# Autodesk Inventor assembly: nc_nhk20
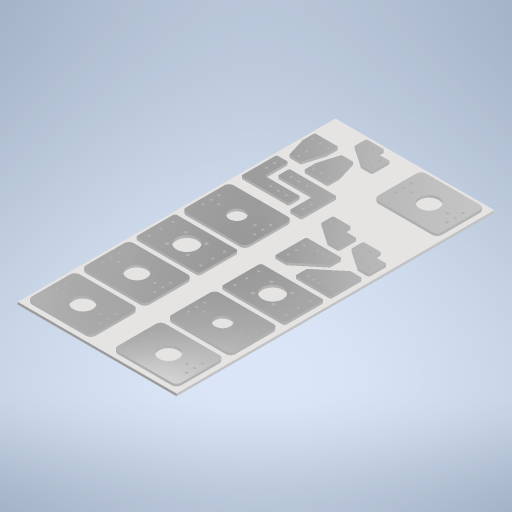
[picture p0: Inventor's stored thumbnail of the model, 512x512]
Saved by Autodesk Inventor 2023 (Build 270158000, 158)
## iProperties
Created: 2022-04-28
Part Number: nc_nhk20
Document SubType Name: Assembly
Designer: yuta
Author: yuta
## Documents named in this file (9)
- C:\Users\yuta\Documents\NHK\nc_nhk20.iam
- C:\Users\yuta\Documents\NHK\NC.port.ipt
- C:\Users\yuta\Documents\NHK\射出_エンコーダー固定.ipt
- C:\Users\yuta\Documents\NHK\射出_エンコーダー固定2.ipt
- C:\Users\yuta\Documents\NHK\射出_モーター固定1.ipt
- C:\Users\yuta\Documents\NHK\射出_固定3.ipt
- C:\Users\yuta\Documents\NHK\射出_固定6.ipt
- C:\Users\yuta\Documents\NHK\射出_固定5.ipt
- C:\Users\yuta\Documents\NHK\射出_固定4.ipt
## Components (18 placed, 8 different names)
1. NC.port:1 — メイト:1, フラッシュ:1, フラッシュ:2, メイト:2, フラッシュ:3, フラッシュ:4, メイト:3, フラッシュ:5, メイト:5, フラッシュ:6, メイト:7, フラッシュ:7, メイト:9, フラッシュ:8, メイト:11, フラッシュ:9, メイト:13, フラッシュ:10, メイト:15, メイト:20, フラッシュ:12, メイト:23, フラッシュ:14, メイト:26, フラッシュ:15, フラッシュ:16, メイト:27, フラッシュ:17, メイト:29, メイト:32, フラッシュ:18, フラッシュ:19
2. 射出_エンコーダー固定:1 — メイト:1, フラッシュ:1, フラッシュ:2, メイト:4
3. 射出_エンコーダー固定:2 — メイト:2, フラッシュ:3, フラッシュ:4, メイト:6
4. 射出_エンコーダー固定:3 — メイト:3, フラッシュ:5, メイト:4, メイト:8
5. 射出_エンコーダー固定2:1 — メイト:11, メイト:12, フラッシュ:9, メイト:21
6. 射出_エンコーダー固定2:2 — メイト:5, メイト:6, フラッシュ:6, メイト:10
7. 射出_モーター固定1:1 — メイト:9, メイト:10, フラッシュ:8, メイト:14, メイト:17
8. 射出_モーター固定1:2 — メイト:7, メイト:8, フラッシュ:7, メイト:12
9. 射出_固定3:1 — メイト:13, メイト:14, フラッシュ:10, メイト:16, メイト:28
10. 射出_固定3:2 — メイト:15, メイト:16, メイト:17, メイト:30
11. 射出_固定6:1 — メイト:18, メイト:19, フラッシュ:11, メイト:20, フラッシュ:12, メイト:24
12. 射出_固定6:2 — メイト:18, メイト:19, フラッシュ:11, メイト:21, メイト:25
13. 射出_固定5:1 — メイト:22, フラッシュ:13, メイト:23, フラッシュ:14, メイト:24
14. 射出_固定5:2 — メイト:22, フラッシュ:13, メイト:25
15. 射出_固定4:1 — メイト:26, フラッシュ:15, フラッシュ:16
16. 射出_固定4:2 — メイト:27, フラッシュ:17, メイト:28, メイト:31
17. 射出_固定4:3 — メイト:29, メイト:30, メイト:31
18. 射出_エンコーダー固定:4 — メイト:32, フラッシュ:18, フラッシュ:19
## Relationships (51: Mate 32, Flush 19)
- メイト:1 [Mate]: NC.port:1 ↔ 射出_エンコーダー固定:1
- フラッシュ:1 [Flush] (6 mm): NC.port:1 ↔ 射出_エンコーダー固定:1
- フラッシュ:2 [Flush] (6 mm): NC.port:1 ↔ 射出_エンコーダー固定:1
- メイト:2 [Mate]: NC.port:1 ↔ 射出_エンコーダー固定:2
- フラッシュ:3 [Flush] (6 mm): NC.port:1 ↔ 射出_エンコーダー固定:2
- フラッシュ:4 [Flush] (6 mm): NC.port:1 ↔ 射出_エンコーダー固定:2
- メイト:3 [Mate]: NC.port:1 ↔ 射出_エンコーダー固定:3
- フラッシュ:5 [Flush] (6 mm): NC.port:1 ↔ 射出_エンコーダー固定:3
- メイト:4 [Mate] (8 mm): 射出_エンコーダー固定:1 ↔ 射出_エンコーダー固定:3
- メイト:5 [Mate]: NC.port:1 ↔ 射出_エンコーダー固定2:2
- メイト:6 [Mate] (8 mm): 射出_エンコーダー固定:2 ↔ 射出_エンコーダー固定2:2
- フラッシュ:6 [Flush] (6 mm): NC.port:1 ↔ 射出_エンコーダー固定2:2
- メイト:7 [Mate]: NC.port:1 ↔ 射出_モーター固定1:2
- メイト:8 [Mate] (8 mm): 射出_エンコーダー固定:3 ↔ 射出_モーター固定1:2
- フラッシュ:7 [Flush] (6 mm): NC.port:1 ↔ 射出_モーター固定1:2
- メイト:9 [Mate]: NC.port:1 ↔ 射出_モーター固定1:1
- メイト:10 [Mate] (8 mm): 射出_エンコーダー固定2:2 ↔ 射出_モーター固定1:1
- フラッシュ:8 [Flush] (6 mm): NC.port:1 ↔ 射出_モーター固定1:1
- メイト:11 [Mate]: NC.port:1 ↔ 射出_エンコーダー固定2:1
- メイト:12 [Mate] (8 mm): 射出_エンコーダー固定2:1 ↔ 射出_モーター固定1:2
- フラッシュ:9 [Flush] (6 mm): NC.port:1 ↔ 射出_エンコーダー固定2:1
- メイト:13 [Mate]: NC.port:1 ↔ 射出_固定3:1
- メイト:14 [Mate] (8 mm): 射出_モーター固定1:1 ↔ 射出_固定3:1
- フラッシュ:10 [Flush] (6 mm): NC.port:1 ↔ 射出_固定3:1
- メイト:15 [Mate]: NC.port:1 ↔ 射出_固定3:2
- メイト:16 [Mate] (8 mm): 射出_固定3:1 ↔ 射出_固定3:2
- メイト:17 [Mate] (17 mm): 射出_モーター固定1:1 ↔ 射出_固定3:2
- メイト:18 [Mate] (8 mm): 射出_固定6:1 ↔ 射出_固定6:2
- メイト:19 [Mate] (8 mm): 射出_固定6:1 ↔ 射出_固定6:2
- フラッシュ:11 [Flush]: 射出_固定6:1 ↔ 射出_固定6:2
- メイト:20 [Mate]: NC.port:1 ↔ 射出_固定6:1
- フラッシュ:12 [Flush] (6 mm): NC.port:1 ↔ 射出_固定6:1
- メイト:21 [Mate] (8 mm): 射出_エンコーダー固定2:1 ↔ 射出_固定6:2
- メイト:22 [Mate] (8 mm): 射出_固定5:1 ↔ 射出_固定5:2
- フラッシュ:13 [Flush]: 射出_固定5:1 ↔ 射出_固定5:2
- メイト:23 [Mate]: NC.port:1 ↔ 射出_固定5:1
- フラッシュ:14 [Flush] (6 mm): NC.port:1 ↔ 射出_固定5:1
- メイト:24 [Mate] (8 mm): 射出_固定6:1 ↔ 射出_固定5:1
- メイト:25 [Mate] (8 mm): 射出_固定6:2 ↔ 射出_固定5:2
- メイト:26 [Mate]: NC.port:1 ↔ 射出_固定4:1
- フラッシュ:15 [Flush] (6 mm): NC.port:1 ↔ 射出_固定4:1
- フラッシュ:16 [Flush] (45 mm): NC.port:1 ↔ 射出_固定4:1
- メイト:27 [Mate]: NC.port:1 ↔ 射出_固定4:2
- フラッシュ:17 [Flush] (6 mm): NC.port:1 ↔ 射出_固定4:2
- メイト:28 [Mate] (8 mm): 射出_固定3:1 ↔ 射出_固定4:2
- メイト:29 [Mate]: NC.port:1 ↔ 射出_固定4:3
- メイト:30 [Mate] (8 mm): 射出_固定3:2 ↔ 射出_固定4:3
- メイト:31 [Mate] (8 mm): 射出_固定4:2 ↔ 射出_固定4:3
- メイト:32 [Mate]: NC.port:1 ↔ 射出_エンコーダー固定:4
- フラッシュ:18 [Flush] (6 mm): NC.port:1 ↔ 射出_エンコーダー固定:4
- フラッシュ:19 [Flush] (6 mm): NC.port:1 ↔ 射出_エンコーダー固定:4
